# Autodesk Inventor assembly: RobotPallet_2
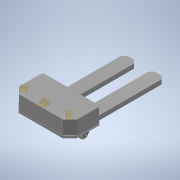
[picture p0: Inventor's stored thumbnail of the model, 180x180]
Saved by Autodesk Inventor 2022.1 (Build 261234000, 234)
## iProperties
Created: 2021-09-10
Part Number: RobotPallet_2
Material: Generic
Document SubType Name: Assembly
Designer: Andres
Author: Andres
## Documents named in this file (9)
- C:\Users\seb_0\Desktop\RobotPallet_v3\RobotPallet_2.iam
- C:\Users\seb_0\Desktop\RobotPallet_v3\Estructura Inferior.iam
- C:\Users\seb_0\Desktop\RobotPallet_v3\plancah base.ipt
- C:\Users\seb_0\Desktop\RobotPallet_v3\apoyo\apoyo2.ipt
- C:\Users\seb_0\Desktop\RobotPallet_v3\Mecanismo de movimiento\Mecanismo - Izquierdo.iam
- C:\Users\seb_0\Desktop\RobotPallet_v3\Mecanismo de movimiento\Mecanismo - Derecho.iam
- C:\Users\seb_0\Desktop\RobotPallet_v3\Horquillas\Horquilla.iam
- C:\Users\seb_0\Desktop\RobotPallet_v3\Carcasa.ipt
- C:\Users\seb_0\Desktop\RobotPallet_v3\LIDARLivox Mid-70.ipt
## Components (14 placed, 8 different names)
1. Estructura Inferior:1 [sub-assembly] — Flush:1, Coincidencia:1, Coincidencia:2, Coincidencia:3, Coincidencia:4, Coincidencia:6, Coincidencia:8, Nivelación:3, Nivelación:4, Nivelación:5, Nivelación:6, Coincidencia:9, Coincidencia:10, Coincidencia:11, Coincidencia:12, Coincidencia:13, Coincidencia:14, Ángulo:1, Ángulo:2, Nivelación:14, Nivelación:15, Nivelación:16
2. planchabase:1 — Flush:1, Nivelación:2, Nivelación:7, Nivelación:8, Nivelación:14, Nivelación:15, Nivelación:16, Coincidencia:22
3. apoyo2:1 — Coincidencia:1, Nivelación:5
4. apoyo2:2 — Coincidencia:2, Coincidencia:5, Nivelación:6
5. apoyo2:3 — Coincidencia:3, Nivelación:4
6. apoyo2:4 — Coincidencia:4, Coincidencia:7, Nivelación:3
7. Mecanismo - Izquierdo:1 [sub-assembly] — Coincidencia:5, Coincidencia:6, Ángulo:2
8. Mecanismo - Derecho:1 [sub-assembly] — Coincidencia:7, Coincidencia:8, Ángulo:1
9. Horquilla:1 [sub-assembly] — Coincidencia:9, Coincidencia:11, Coincidencia:13
10. Horquilla:2 [sub-assembly] — Coincidencia:10, Coincidencia:12, Coincidencia:14
11. Carcasa:1 — Nivelación:7, Nivelación:8, Nivelación:11, Coincidencia:18, Ángulo:3, Nivelación:12, Coincidencia:19, Ángulo:4, Nivelación:13, Coincidencia:20, Coincidencia:21, Coincidencia:22, Nivelación:17, Coincidencia:23
12. LIDARLivox Mid-70:1 — Nivelación:11, Nivelación:17, Coincidencia:23
13. LIDARLivox Mid-70:2 — Coincidencia:18, Ángulo:3, Nivelación:12, Coincidencia:20
14. LIDARLivox Mid-70:3 — Coincidencia:19, Ángulo:4, Nivelación:13, Coincidencia:21
## Relationships (39: Mate 20, Flush 15, Angle 4)
- Flush:1: Estructura Inferior:1 ↔ planchabase:1
- Nivelación:2 [Flush]: planchabase:1
- Coincidencia:1 [Mate]: Estructura Inferior:1 ↔ apoyo2:1
- Coincidencia:2 [Mate]: Estructura Inferior:1 ↔ apoyo2:2
- Coincidencia:3 [Mate]: Estructura Inferior:1 ↔ apoyo2:3
- Coincidencia:4 [Mate]: Estructura Inferior:1 ↔ apoyo2:4
- Coincidencia:5 [Mate]: apoyo2:2 ↔ Mecanismo - Izquierdo:1
- Coincidencia:6 [Mate] (2.5 mm): Estructura Inferior:1 ↔ Mecanismo - Izquierdo:1
- Coincidencia:7 [Mate]: apoyo2:4 ↔ Mecanismo - Derecho:1
- Coincidencia:8 [Mate] (2.5 mm): Estructura Inferior:1 ↔ Mecanismo - Derecho:1
- Nivelación:3 [Flush] (180 mm): Estructura Inferior:1 ↔ apoyo2:4
- Nivelación:4 [Flush] (180 mm): Estructura Inferior:1 ↔ apoyo2:3
- Nivelación:5 [Flush] (180 mm): Estructura Inferior:1 ↔ apoyo2:1
- Nivelación:6 [Flush] (180 mm): Estructura Inferior:1 ↔ apoyo2:2
- Coincidencia:9 [Mate]: Estructura Inferior:1 ↔ Horquilla:1
- Coincidencia:10 [Mate]: Estructura Inferior:1 ↔ Horquilla:2
- Coincidencia:11 [Mate]: Estructura Inferior:1 ↔ Horquilla:1
- Coincidencia:12 [Mate]: Estructura Inferior:1 ↔ Horquilla:2
- Coincidencia:13 [Mate] (-100 mm): Estructura Inferior:1 ↔ Horquilla:1
- Coincidencia:14 [Mate] (-100 mm): Estructura Inferior:1 ↔ Horquilla:2
- Ángulo:1 [Angle] (0 deg): Estructura Inferior:1 ↔ Mecanismo - Derecho:1
- Ángulo:2 [Angle] (180 deg): Estructura Inferior:1 ↔ Mecanismo - Izquierdo:1
- Nivelación:7 [Flush]: planchabase:1 ↔ Carcasa:1
- Nivelación:8 [Flush]: planchabase:1 ↔ Carcasa:1
- Nivelación:11 [Flush] (404 mm): Carcasa:1 ↔ LIDARLivox Mid-70:1
- Coincidencia:18 [Mate]: Carcasa:1 ↔ LIDARLivox Mid-70:2
- Ángulo:3 [Angle] (180 deg): Carcasa:1 ↔ LIDARLivox Mid-70:2
- Nivelación:12 [Flush]: Carcasa:1 ↔ LIDARLivox Mid-70:2
- Coincidencia:19 [Mate]: Carcasa:1 ↔ LIDARLivox Mid-70:3
- Ángulo:4 [Angle] (180 deg): Carcasa:1 ↔ LIDARLivox Mid-70:3
- Nivelación:13 [Flush]: Carcasa:1 ↔ LIDARLivox Mid-70:3
- Nivelación:14 [Flush] (4 mm): Estructura Inferior:1 ↔ planchabase:1
- Nivelación:15 [Flush] (-4 mm): Estructura Inferior:1 ↔ planchabase:1
- Nivelación:16 [Flush] (-4 mm): Estructura Inferior:1 ↔ planchabase:1
- Coincidencia:20 [Mate] (40 mm): Carcasa:1 ↔ LIDARLivox Mid-70:2
- Coincidencia:21 [Mate] (40 mm): Carcasa:1 ↔ LIDARLivox Mid-70:3
- Coincidencia:22 [Mate]: planchabase:1 ↔ Carcasa:1
- Nivelación:17 [Flush]: Carcasa:1 ↔ LIDARLivox Mid-70:1
- Coincidencia:23 [Mate]: Carcasa:1 ↔ LIDARLivox Mid-70:1
